# Autodesk Inventor assembly: screw_lift_left
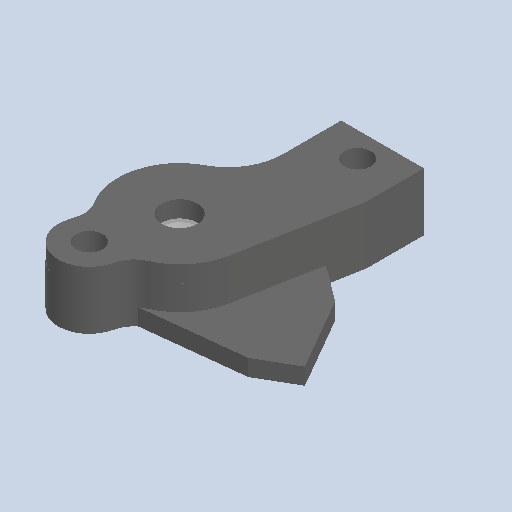
[picture p0: Inventor's stored thumbnail of the model, 512x512]
Saved by Autodesk Inventor 2024.1 (Build 281209000, 209)
## iProperties
Created: 2025-01-18
Part Number: screw_lift_left
Document SubType Name: Assembly
Designer: hibik
Author: hibik
## Documents named in this file (4)
- C:\Users\hibik\Documents\Robomech\RESCUE\ORCA\hard\fork\left\screw_lift_left.iam
- C:\Users\hibik\Documents\Robomech\RESCUE\ORCA\hard\fork\left\nat_M4_left.ipt
- C:\Users\hibik\Documents\Robomech\RESCUE\ORCA\hard\fork\left\screw_lift_under_left.ipt
- C:\Users\hibik\Documents\Robomech\RESCUE\ORCA\hard\fork\left\screw_lift_upper_left.ipt
## Components (3 placed, 3 different names)
1. nat_M4_left:1 — 角度:1, 挿入:1
2. screw_lift_under_left:1 — 角度:1, 挿入:1, メイト:1, フラッシュ:2, フラッシュ:1
3. screw_lift_upper_left:1 — メイト:1, フラッシュ:2, フラッシュ:1
## Relationships (5: Flush 2, Angle 1, Insert 1, Mate 1)
- 角度:1 [Angle] (0 deg): nat_M4_left:1 ↔ screw_lift_under_left:1
- 挿入:1 [Insert]: nat_M4_left:1 ↔ screw_lift_under_left:1
- メイト:1 [Mate]: screw_lift_under_left:1 ↔ screw_lift_upper_left:1
- フラッシュ:2 [Flush]: screw_lift_under_left:1 ↔ screw_lift_upper_left:1
- フラッシュ:1 [Flush]: screw_lift_under_left:1 ↔ screw_lift_upper_left:1
